# Autodesk Inventor assembly: driveAssembly_MIR1
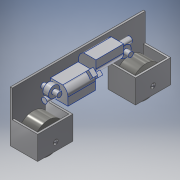
[picture p0: Inventor's stored thumbnail of the model, 180x180]
Saved by Autodesk Inventor 2016 (Build 200138000, 138)
## iProperties
Created: 2015-10-31
Part Number: driveAssembly_MIR1
Document SubType Name: Assembly
Designer: rossmosier
Author: rossmosier
## Documents named in this file (6)
- C:\Users\rossmosier\Documents\CAD Team\CADTeam\Drive Train\driveAssembly_MIR1.iam
- C:\Users\rossmosier\Documents\CAD Team\CADTeam\Drive Train\side_MIR1.ipt
- C:\Users\rossmosier\Documents\CAD Team\CADTeam\Drive Train\driveAssembly\Design Accelerator\Shaft1_MIR1.iam
- C:\Users\rossmosier\Documents\CAD Team\CADTeam\Parts\bearing_MIR1.ipt
- C:\Users\rossmosier\Documents\CAD Team\CADTeam\Drive Train\generic wheel_MIR1.ipt
- C:\Users\rossmosier\Documents\CAD Team\CADTeam\Drive Train\Motor_500RPM_MIR.ipt
## Components (9 placed, 5 different names)
1. side_MIR1:1 — Mate:1, Mate:2
2. Shaft1_MIR1:1 [sub-assembly] — Rotational:2, Rotational:4
3. bearing_MIR1:1 — Rotational:2
4. bearing_MIR1:2 — Rotational:3
5. Shaft1_MIR1:2 [sub-assembly] — Rotational:3
6. generic wheel_MIR1:1
7. generic wheel_MIR1:2 — Rotational:4
8. Motor_500RPM_MIR:1 — Mate:1
9. Motor_500RPM_MIR:2 — Mate:2
## Relationships (5: RevoluteJoint 3, Mate 2)
- Mate:1: side_MIR1:1 ↔ Motor_500RPM_MIR:1
- Mate:2: side_MIR1:1 ↔ Motor_500RPM_MIR:2
- Rotational:2 [RevoluteJoint] (6.35 mm): Shaft1_MIR1:1 ↔ bearing_MIR1:1
- Rotational:3 [RevoluteJoint] (6.35 mm): bearing_MIR1:2 ↔ Shaft1_MIR1:2
- Rotational:4 [RevoluteJoint] (25.4 mm): Shaft1_MIR1:1 ↔ generic wheel_MIR1:2
